# Autodesk Inventor assembly: base_assembly
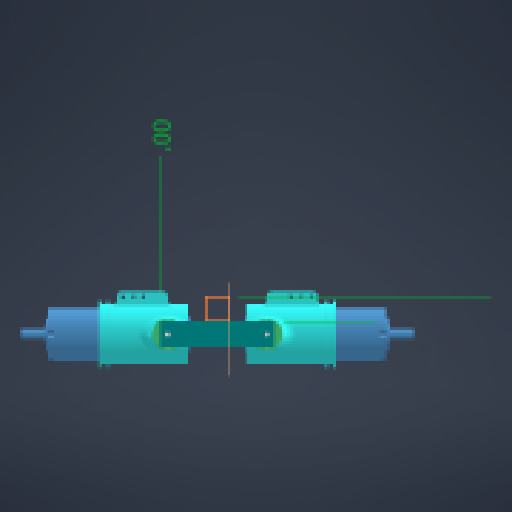
[picture p0: Inventor's stored thumbnail of the model, 512x512]
Saved by Autodesk Inventor 2024 (Build 280153000, 153)
## iProperties
Created: 2023-04-14
Part Number: base_assembly
Document SubType Name: Assembly
Designer: user
Author: user
## Documents named in this file (8)
- D:\DOC\Robot\3d\base\base_assembly.iam
- D:\DOC\Robot\3d\base\main axis.ipt
- D:\DOC\Robot\3d\base\section.ipt
- D:\DOC\Robot\3d\motor_assembly\side\motor_assembly_S.iam
- D:\DOC\Robot\3d\motor_assembly\side\motor_assembly_S_MIR.iam
- D:\DOC\Robot\3d\motor_assembly\midel\motor_assembly_M.iam
- D:\DOC\Robot\3d\base\arm.ipt
- D:\DOC\Robot\3d\default_components\shock_absorber.ipt
## Components (20 placed, 7 different names)
1. main axis:1 — Совмещение:1, Совмещение:2, Угол:1, Совмещение:8, Жесткий:1, Жесткий:5
2. section:1 — Совмещение:1, Совмещение:2, Вставка:2, Вставка:3
3. section:3 — Вставка:4, Вставка:5, Вставка:6, Вставка:7
4. motor_assembly_M:1 [sub-assembly] — Вставка:6, Вставка:9, Совмещение:4
5. motor_assembly_M:2 [sub-assembly] — Вставка:7, Вставка:8, Совмещение:6
6. motor_assembly_S:1 [sub-assembly] — Вставка:3, Вставка:5, Совмещение:5
7. motor_assembly_S_MIR:1 [sub-assembly] — Вставка:2, Вставка:4, Совмещение:7
8. section:4 — Вставка:8, Вставка:9, Вставка:10, Вставка:14
9. section:5 — Вставка:13, Вставка:15
10. motor_assembly_S:2 [sub-assembly] — Вставка:10, Вставка:13, Совмещение:3, Совмещение:6, Совмещение:7, Вставка:16
11. motor_assembly_S_MIR:2 [sub-assembly] — Вставка:14, Вставка:15, Угол:1, Совмещение:3, Совмещение:4, Совмещение:5
12. arm:1 — Жесткий:1, Жесткий:2
13. arm:2 — Жесткий:2, Жесткий:3
14. arm:3 — Жесткий:3, Жесткий:4
15. arm:4 — Жесткий:4
16. arm:5 — Жесткий:5, Жесткий:6
17. arm:6 — Жесткий:6, Жесткий:7
18. arm:7 — Жесткий:7, Жесткий:8
19. arm:8 — Жесткий:8
20. shock_absorber:1 — Вставка:16
## Relationships (31: Insert 13, Mate 8, WeldJoint 8, Angle 2)
- Совмещение:1 [Mate]: main axis:1 ↔ section:1
- Совмещение:2 [Mate] (55 mm): main axis:1 ↔ section:1
- Вставка:2 [Insert]: section:1 ↔ motor_assembly_S_MIR:1
- Вставка:3 [Insert]: section:1 ↔ motor_assembly_S:1
- Вставка:4 [Insert]: section:3 ↔ motor_assembly_S_MIR:1
- Вставка:5 [Insert]: section:3 ↔ motor_assembly_S:1
- Вставка:6 [Insert]: section:3 ↔ motor_assembly_M:1
- Вставка:7 [Insert]: section:3 ↔ motor_assembly_M:2
- Вставка:8 [Insert]: motor_assembly_M:2 ↔ section:4
- Вставка:9 [Insert]: motor_assembly_M:1 ↔ section:4
- Вставка:10 [Insert]: section:4 ↔ motor_assembly_S:2
- Вставка:13 [Insert]: section:5 ↔ motor_assembly_S:2
- Вставка:14 [Insert]: section:4 ↔ motor_assembly_S_MIR:2
- Вставка:15 [Insert]: section:5 ↔ motor_assembly_S_MIR:2
- Угол:1 [Angle] (0 deg): main axis:1 ↔ motor_assembly_S_MIR:2
- Совмещение:3 [Mate]: motor_assembly_S:2 ↔ motor_assembly_S_MIR:2
- Совмещение:4 [Mate]: motor_assembly_M:1 ↔ motor_assembly_S_MIR:2
- Совмещение:5 [Mate]: motor_assembly_S:1 ↔ motor_assembly_S_MIR:2
- Совмещение:6 [Mate]: motor_assembly_M:2 ↔ motor_assembly_S:2
- Совмещение:7 [Mate]: motor_assembly_S_MIR:1 ↔ motor_assembly_S:2
- Совмещение:8 [Mate]: main axis:1
- Угол:2 [Angle] (0 deg)
- Жесткий:1 [WeldJoint]: main axis:1 ↔ arm:1
- Жесткий:2 [WeldJoint] (-126 mm): arm:1 ↔ arm:2
- Жесткий:3 [WeldJoint] (140 mm): arm:2 ↔ arm:3
- Жесткий:4 [WeldJoint] (106 mm): arm:3 ↔ arm:4
- Жесткий:5 [WeldJoint]: main axis:1 ↔ arm:5
- Жесткий:6 [WeldJoint] (106 mm): arm:5 ↔ arm:6
- Жесткий:7 [WeldJoint] (140 mm): arm:6 ↔ arm:7
- Жесткий:8 [WeldJoint] (106 mm): arm:7 ↔ arm:8
- Вставка:16 [Insert]: motor_assembly_S:2 ↔ shock_absorber:1
## Named parameters: hw = 1 mm
